# Autodesk Inventor assembly: base_assem
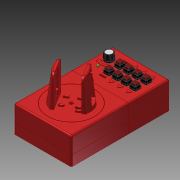
[picture p0: Inventor's stored thumbnail of the model, 180x180]
Saved by Autodesk Inventor 2014 (Build 180170000, 170)
## iProperties
Created: 2014-04-22
Part Number: base_assem
Document SubType Name: Assembly
Designer: t_emanb
Author: t_emanb
## Documents named in this file (14)
- C:\Users\t_emanb\Documents\3D printed arm\4th version\base_assem.iam
- C:\Users\t_emanb\Documents\3D printed arm\4th version\base_bottombuttonsBox.ipt
- C:\Users\t_emanb\Documents\3D printed arm\4th version\base_bottomrotateBox.ipt
- C:\Users\t_emanb\Documents\3D printed arm\4th version\base_topbuttonsBox.ipt
- C:\Users\t_emanb\Documents\3D printed arm\4th version\base_toprotateBox.ipt
- C:\Users\t_emanb\Documents\3D printed arm\4th version\base_bottomrotate.ipt
- C:\Users\t_emanb\Documents\3D printed arm\4th version\base_toprotate.ipt
- C:\Users\t_emanb\Documents\3D printed arm\stock parts\servo_assem.iam
- C:\Users\t_emanb\Documents\3D printed arm\stock parts\arduino_uno.ipt
- C:\Users\t_emanb\Documents\3D printed arm\stock parts\pushbutton_2751566.ipt
- C:\Users\t_emanb\Documents\3D printed arm\stock parts\led.ipt
- C:\Users\t_emanb\Documents\3D printed arm\4th version\base_servomountcurve.ipt
- C:\Users\t_emanb\Documents\3D printed arm\4th version\base_servomountcurveMirror.ipt
- C:\Users\t_emanb\Documents\3D printed arm\stock parts\knob_pot.ipt
## Components (20 placed, 13 different names)
1. base_bottombuttonsBox:1 — Flush:1, Mate:1, Flush:2, Flush:7, Mate:2
2. base_bottomrotateBox:1 — Flush:1, Mate:1, Flush:2, Flush:5, Flush:6, Mate:18
3. base_topbuttonsBox:1 — Flush:3, Flush:4, Flush:5, Flush:6, Mate:19, Mate:20, Mate:21, Mate:22, Mate:23, Mate:24, Mate:25, Mate:26, Mate:27, Mate:28, Mate:29, Mate:30, Mate:31, Mate:32, Mate:33, Mate:34, Mate:35, Mate:36, Mate:37, Mate:38, Mate:39, Mate:40, Mate:47, Mate:48, Mate:52, Mate:53, Mate:54, Mate:55, Mate:56, Mate:57
4. base_toprotateBox:1 — Flush:3, Flush:4, Flush:7, Mate:2, Flush:8, Angle:1, Mate:49
5. base_bottomrotate:1 — Mate:5, Mate:13, Mate:14, Mate:50, Mate:51
6. base_toprotate:1 — Mate:5, Flush:8, Mate:15, Mate:41, Mate:42, Mate:43, Mate:44, Mate:45, Mate:46, Mate:49, Mate:50, Mate:51
7. servo_assem:1 [sub-assembly] — Mate:13, Mate:14, Mate:15, Angle:1
8. arduino_uno:1 — Mate:18
9. pushbutton_2751566:1 — Mate:19, Mate:31, Mate:32
10. pushbutton_2751566:2 — Mate:20, Mate:36, Mate:37, Mate:38
11. pushbutton_2751566:3 — Mate:21, Mate:26, Mate:28
12. pushbutton_2751566:4 — Mate:22, Mate:29, Mate:30
13. pushbutton_2751566:5 — Mate:23, Mate:33, Mate:34, Mate:35
14. pushbutton_2751566:6 — Mate:24, Mate:25, Mate:27
15. led:1 — Mate:39, Mate:40
16. base_servomountcurve:1 — Mate:41, Mate:42, Mate:43
17. base_servomountcurveMirror:1 — Mate:44, Mate:45, Mate:46
18. knob_pot:1 — Mate:47, Mate:48
19. pushbutton_2751566:7 — Mate:52, Mate:54, Mate:57
20. pushbutton_2751566:8 — Mate:53, Mate:55, Mate:56
## Relationships (55: Mate 46, Flush 8, Angle 1)
- Flush:1: base_bottombuttonsBox:1 ↔ base_bottomrotateBox:1
- Mate:1: base_bottombuttonsBox:1 ↔ base_bottomrotateBox:1
- Flush:2: base_bottombuttonsBox:1 ↔ base_bottomrotateBox:1
- Flush:3: base_topbuttonsBox:1 ↔ base_toprotateBox:1
- Flush:4: base_topbuttonsBox:1 ↔ base_toprotateBox:1
- Flush:5: base_bottomrotateBox:1 ↔ base_topbuttonsBox:1
- Flush:6: base_bottomrotateBox:1 ↔ base_topbuttonsBox:1
- Flush:7: base_bottombuttonsBox:1 ↔ base_toprotateBox:1
- Mate:2: base_bottombuttonsBox:1 ↔ base_toprotateBox:1
- Mate:5: base_bottomrotate:1 ↔ base_toprotate:1
- Flush:8: base_toprotateBox:1 ↔ base_toprotate:1
- Mate:13: base_bottomrotate:1 ↔ servo_assem:1
- Mate:14: base_bottomrotate:1 ↔ servo_assem:1
- Mate:15: base_toprotate:1 ↔ servo_assem:1
- Angle:1 (0 deg): base_toprotateBox:1 ↔ servo_assem:1
- Mate:18 (2.032 mm): base_bottomrotateBox:1 ↔ arduino_uno:1
- Mate:19: base_topbuttonsBox:1 ↔ pushbutton_2751566:1
- Mate:20: base_topbuttonsBox:1 ↔ pushbutton_2751566:2
- Mate:21: base_topbuttonsBox:1 ↔ pushbutton_2751566:3
- Mate:22: base_topbuttonsBox:1 ↔ pushbutton_2751566:4
- Mate:23: base_topbuttonsBox:1 ↔ pushbutton_2751566:5
- Mate:24: base_topbuttonsBox:1 ↔ pushbutton_2751566:6
- Mate:25: base_topbuttonsBox:1 ↔ pushbutton_2751566:6
- Mate:26: base_topbuttonsBox:1 ↔ pushbutton_2751566:3
- Mate:27: base_topbuttonsBox:1 ↔ pushbutton_2751566:6
- Mate:28: base_topbuttonsBox:1 ↔ pushbutton_2751566:3
- Mate:29: base_topbuttonsBox:1 ↔ pushbutton_2751566:4
- Mate:30: base_topbuttonsBox:1 ↔ pushbutton_2751566:4
- Mate:31: base_topbuttonsBox:1 ↔ pushbutton_2751566:1
- Mate:32: base_topbuttonsBox:1 ↔ pushbutton_2751566:1
- Mate:33: base_topbuttonsBox:1 ↔ pushbutton_2751566:5
- Mate:34: base_topbuttonsBox:1 ↔ pushbutton_2751566:5
- Mate:35: base_topbuttonsBox:1 ↔ pushbutton_2751566:5
- Mate:36: base_topbuttonsBox:1 ↔ pushbutton_2751566:2
- Mate:37: base_topbuttonsBox:1 ↔ pushbutton_2751566:2
- Mate:38: base_topbuttonsBox:1 ↔ pushbutton_2751566:2
- Mate:39: base_topbuttonsBox:1 ↔ led:1
- Mate:40: base_topbuttonsBox:1 ↔ led:1
- Mate:41: base_toprotate:1 ↔ base_servomountcurve:1
- Mate:42: base_toprotate:1 ↔ base_servomountcurve:1
- Mate:43: base_toprotate:1 ↔ base_servomountcurve:1
- Mate:44: base_toprotate:1 ↔ base_servomountcurveMirror:1
- Mate:45: base_toprotate:1 ↔ base_servomountcurveMirror:1
- Mate:46: base_toprotate:1 ↔ base_servomountcurveMirror:1
- Mate:47: base_topbuttonsBox:1 ↔ knob_pot:1
- Mate:48: base_topbuttonsBox:1 ↔ knob_pot:1
- Mate:49: base_toprotateBox:1 ↔ base_toprotate:1
- Mate:50: base_bottomrotate:1 ↔ base_toprotate:1
- Mate:51: base_bottomrotate:1 ↔ base_toprotate:1
- Mate:52: base_topbuttonsBox:1 ↔ pushbutton_2751566:7
- Mate:53: base_topbuttonsBox:1 ↔ pushbutton_2751566:8
- Mate:54: base_topbuttonsBox:1 ↔ pushbutton_2751566:7
- Mate:55: base_topbuttonsBox:1 ↔ pushbutton_2751566:8
- Mate:56: base_topbuttonsBox:1 ↔ pushbutton_2751566:8
- Mate:57: base_topbuttonsBox:1 ↔ pushbutton_2751566:7
